# Autodesk Inventor assembly: Kermit Bumper 4
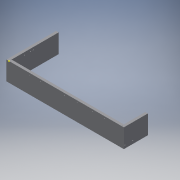
[picture p0: Inventor's stored thumbnail of the model, 180x180]
Saved by Autodesk Inventor 2018.2 (Build 222227000, 227)
## iProperties
Created: 2018-02-17
Part Number: Kermit Bumper 4
Document SubType Name: Assembly
Designer: lopez.xavier
Author: lopez.xavier
## Documents named in this file (4)
- \\fs1\studentusers\class19\Lopez.Xavier\documents\Cad\Cad-Team-J-\Kermit Bumper 4.iam
- C:\Users\lopez.xavier.NICHOLSNT.001\Downloads\kermit_bumper_Medium_4.ipt
- C:\Users\lopez.xavier.NICHOLSNT.001\Downloads\Kermit_bumper_middle_4.ipt
- C:\Users\lopez.xavier.NICHOLSNT.001\Downloads\kermit_bumper_small_4.ipt
## Components (3 placed, 3 different names)
1. kermit_bumper_Medium_4:1 — Flush:3, Flush:4, Mate:2
2. Kermit_bumper_middle_4:1 — Flush:1, Mate:1, Flush:2, Flush:3, Flush:4, Mate:2
3. kermit_bumper_small_4:1 — Flush:1, Mate:1, Flush:2
## Relationships (6: Flush 4, Mate 2)
- Flush:1: Kermit_bumper_middle_4:1 ↔ kermit_bumper_small_4:1
- Mate:1: Kermit_bumper_middle_4:1 ↔ kermit_bumper_small_4:1
- Flush:2: Kermit_bumper_middle_4:1 ↔ kermit_bumper_small_4:1
- Flush:3: kermit_bumper_Medium_4:1 ↔ Kermit_bumper_middle_4:1
- Flush:4: kermit_bumper_Medium_4:1 ↔ Kermit_bumper_middle_4:1
- Mate:2: kermit_bumper_Medium_4:1 ↔ Kermit_bumper_middle_4:1
